# Autodesk Inventor assembly: Piston Assembly
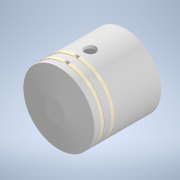
[picture p0: Inventor's stored thumbnail of the model, 180x180]
Saved by Autodesk Inventor 2020 (Build 240168000, 168)
## iProperties
Created: 2020-08-09
Part Number: Piston Assembly
Document SubType Name: Assembly
Designer: benny
Author: benny
## Documents named in this file (4)
- C:\Users\benny\Desktop\importantmajorprojecthev_june\engine\piston assembly\Piston Assembly.iam
- C:\Users\benny\Desktop\importantmajorprojecthev_june\engine\piston assembly\piston.ipt
- C:\Users\benny\Desktop\importantmajorprojecthev_june\engine\piston assembly\piston compression ring.ipt
- C:\Users\benny\Documents\Inventor\Content Center Files\R2020\en-US\ISO 2338(2)\ISO 2338 - 5 h8 x 30.ipt
## Components (4 placed, 3 different names)
1. piston:1 — Mate:1, Mate:2, Mate:3, Mate:4, Mate:5
2. piston compression ring:1 — Mate:2
3. piston compression ring:2 — Mate:1, Mate:3
4. ISO 2338 5 h8 x 30:1 — Mate:4, Mate:5
## Relationships (5: Mate 5)
- Mate:1: piston:1 ↔ piston compression ring:2
- Mate:2: piston:1 ↔ piston compression ring:1
- Mate:3: piston:1 ↔ piston compression ring:2
- Mate:4: piston:1 ↔ ISO 2338 5 h8 x 30:1
- Mate:5 (-14.75 mm): piston:1 ↔ ISO 2338 5 h8 x 30:1
